# Autodesk Inventor assembly: Link4
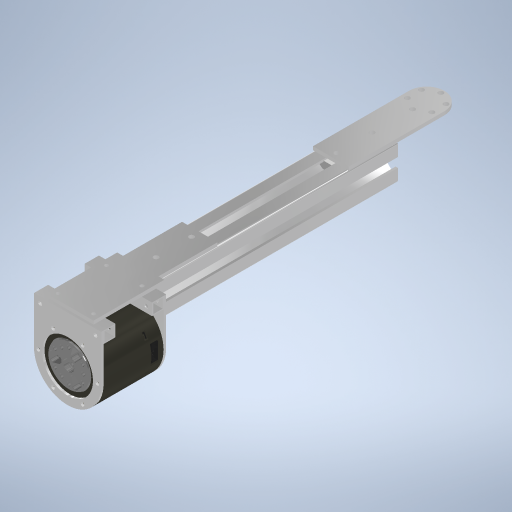
[picture p0: Inventor's stored thumbnail of the model, 512x512]
Saved by Autodesk Inventor 2024 (Build 280153000, 153)
## iProperties
Created: 2024-12-13
Part Number: Link4
Document SubType Name: Assembly
Designer: hirek
Mass: 381.567 g
Surface Area: 776.395 cm^2
Volume: 68.2473 cm^3
Density: 5.59095 g/cm^3
Author: hirek
## Documents named in this file (9)
- E:\Documents\Inventor\CanAloha\Link4.iam
- E:\Documents\Inventor\CanAloha\myperts\link4_plate1.ipt
- E:\Documents\Inventor\CanAloha\official\robStride00\robStride00.iam
- E:\Documents\Inventor\CanAloha\myperts\link4_plate2.ipt
- E:\Documents\Inventor\CanAloha\myperts\link4_plate3.ipt
- E:\Documents\Inventor\CanAloha\myperts\link4_pipe1.ipt
- E:\Documents\Inventor\CanAloha\official\NFSL6-3030-500\NFSL6-3030-500.ipt
- E:\Documents\Inventor\CanAloha\myperts\link4_plate4.ipt
- E:\Documents\Inventor\CanAloha\official\HNTT6-4\AIS2024\HNTT6-4.ipt
## Components (12 placed, 8 different names)
1. link4_plate1:1 — 回転:19, 回転:20, 回転:26, 回転:27
2. robStride00:1 [sub-assembly] — 回転:11, 回転:12, 回転:13, 回転:14
3. link4_plate2:1 — 回転:11, 回転:12, 回転:15, 回転:16, メイト:9
4. link4_plate3:1 — 回転:13, 回転:14, 回転:17, 回転:18
5. link4_pipe1:1 — 回転:15, 回転:16, 回転:20
6. link4_pipe1:2 — 回転:17, 回転:18, 回転:19
7. NFSL6-3030-500:1 — メイト:1, メイト:2, メイト:3, メイト:4, メイト:5, メイト:6, メイト:7, メイト:8, メイト:9, フラッシュ:1
8. link4_plate4:1 — 回転:22, 回転:25
9. HNTT6-4:1 — メイト:1, メイト:6, 回転:27
10. HNTT6-4:2 — メイト:2, メイト:7, 回転:22
11. HNTT6-4:3 — メイト:3, メイト:8, フラッシュ:1, 回転:25
12. HNTT6-4:4 — メイト:4, メイト:5, 回転:26
## Relationships (24: RevoluteJoint 14, Mate 9, Flush 1)
- 回転:11 [RevoluteJoint]: robStride00:1 ↔ link4_plate2:1
- 回転:12 [RevoluteJoint]: robStride00:1 ↔ link4_plate2:1
- 回転:13 [RevoluteJoint]: robStride00:1 ↔ link4_plate3:1
- 回転:14 [RevoluteJoint]: robStride00:1 ↔ link4_plate3:1
- 回転:15 [RevoluteJoint]: link4_plate2:1 ↔ link4_pipe1:1
- 回転:16 [RevoluteJoint]: link4_plate2:1 ↔ link4_pipe1:1
- 回転:17 [RevoluteJoint]: link4_plate3:1 ↔ link4_pipe1:2
- 回転:18 [RevoluteJoint]: link4_plate3:1 ↔ link4_pipe1:2
- 回転:19 [RevoluteJoint]: link4_plate1:1 ↔ link4_pipe1:2
- 回転:20 [RevoluteJoint]: link4_plate1:1 ↔ link4_pipe1:1
- メイト:1 [Mate]: NFSL6-3030-500:1 ↔ HNTT6-4:1
- メイト:2 [Mate]: NFSL6-3030-500:1 ↔ HNTT6-4:2
- メイト:3 [Mate]: NFSL6-3030-500:1 ↔ HNTT6-4:3
- メイト:4 [Mate]: NFSL6-3030-500:1 ↔ HNTT6-4:4
- メイト:5 [Mate]: NFSL6-3030-500:1 ↔ HNTT6-4:4
- メイト:6 [Mate]: NFSL6-3030-500:1 ↔ HNTT6-4:1
- メイト:7 [Mate]: NFSL6-3030-500:1 ↔ HNTT6-4:2
- メイト:8 [Mate]: NFSL6-3030-500:1 ↔ HNTT6-4:3
- 回転:22 [RevoluteJoint] (-1.2 mm): link4_plate4:1 ↔ HNTT6-4:2
- メイト:9 [Mate]: link4_plate2:1 ↔ NFSL6-3030-500:1
- フラッシュ:1 [Flush]: NFSL6-3030-500:1 ↔ HNTT6-4:3
- 回転:25 [RevoluteJoint] (-1.2 mm): link4_plate4:1 ↔ HNTT6-4:3
- 回転:26 [RevoluteJoint] (-1.2 mm): link4_plate1:1 ↔ HNTT6-4:4
- 回転:27 [RevoluteJoint] (-1.2 mm): link4_plate1:1 ↔ HNTT6-4:1
